# Autodesk Inventor assembly: BombaPerisImprimible
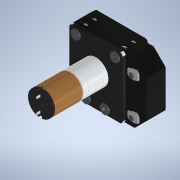
[picture p0: Inventor's stored thumbnail of the model, 180x180]
Saved by Autodesk Inventor 2020.2 (Build 242310000, 310)
## iProperties
Created: 2020-12-04
Part Number: BombaPerisImprimible
Document SubType Name: Assembly
Designer: JK
Sending System: Autodesk Inventor 2020
Preprocessor: ST-DEVELOPER v18
Title: D:\Desk\Drés\2020\Trabajo personal\jk\Podasana\bomba peristaltica\imp\BombaPerisImprimible.stp
Author: andre
## Documents named in this file (12)
- C:\Users\JK\Documents\Inventor\BioMixer\BombaPeristaltica\BombaPeristaltica.iam
- C:\Users\JK\Documents\Inventor\BioMixer\BombaPeristaltica\Impulsor.iam
- C:\Users\JK\Documents\Inventor\BioMixer\BombaPeristaltica\Caja.ipt
- C:\Users\JK\Documents\Inventor\BioMixer\BombaPeristaltica\TapaInferior.ipt
- C:\Users\JK\Documents\Inventor\BioMixer\BombaPeristaltica\TapaSuperior.ipt
- C:\Users\JK\Documents\Inventor\BioMixer\BombaPeristaltica\PernoM3x6Avellanado.ipt
- C:\Users\JK\Documents\Inventor\BioMixer\BombaPeristaltica\PernoM5x25Plano.ipt
- C:\Users\JK\Documents\Inventor\BioMixer\BombaPeristaltica\PernoM5x10Plano.ipt
- C:\Users\JK\Documents\Inventor\BioMixer\BombaPeristaltica\TuercaTM5Perfil2020.ipt
- C:\Users\JK\Documents\Inventor\BioMixer\BombaPeristaltica\MotorDC12V100RPM.ipt
- C:\Users\JK\Documents\Inventor\BioMixer\BombaPeristaltica\TuercaM5.ipt
- C:\Users\JK\Documents\Inventor\BioMixer\BombaPeristaltica\GolillaM5DIN125.ipt
## Components (28 placed, 11 different names)
1. MotorDC12V100RPM:1
2. Impulsor [sub-assembly] — Mate:67
3. Caja — Mate:3, Mate:4, Mate:16, Mate:19, Mate:24, Mate:25, Mate:26, Mate:27, Mate:35, Mate:48, Mate:49, Mate:50, Mate:51, Mate:52, Mate:53, Mate:54, Mate:55, Mate:56, Angle:1
4. TapaSuperior — Mate:3, Mate:4, Mate:38, Mate:39, Mate:40, Mate:41, Mate:42
5. PernoM5x10Plano:1 — Flush:13, Flush:14, Mate:40, Mate:58
6. PernoM5x10Plano:2 — Flush:13, Mate:41, Mate:42, Mate:60
7. PernoM5x10Plano:3 — Flush:15, Mate:38, Mate:56, Mate:63
8. PernoM5x10Plano:4 — Flush:14, Flush:15, Mate:39, Mate:62
9. PernoM5x10Plano:5 — Flush:17, Flush:18, Mate:43, Mate:44, Mate:59
10. PernoM5x10Plano:6 — Flush:17, Mate:45, Mate:57
11. PernoM5x10Plano:7 — Flush:16, Mate:47, Mate:64
12. PernoM5x10Plano:8 — Flush:16, Flush:18, Mate:46, Mate:61
13. PernoM3x6Avellanado:1 — Flush:10
14. TapaInferior:1 — Mate:16, Mate:19, Flush:12, Mate:43, Mate:44, Mate:45, Mate:46, Mate:47, Mate:66
15. PernoM5x25Plano:1 — Mate:25, Mate:26, Mate:29, Flush:9
16. PernoM5x25Plano:2 — Mate:24, Mate:27, Mate:28, Flush:9
17. TuercaTM5Perfil2020:1 — Mate:28, Flush:8, Flush:11
18. TuercaTM5Perfil2020:2 — Mate:29, Flush:8, Mate:35, Flush:11
19. PernoM3x6Avellanado:2 — Flush:10, Flush:12
20. TuercaM5:1 — Mate:48, Angle:7, Mate:63
21. TuercaM5:2 — Mate:49, Angle:5, Mate:62
22. TuercaM5:3 — Mate:50, Angle:5, Angle:6, Mate:61
23. TuercaM5:4 — Mate:51, Angle:6, Angle:7, Mate:64
24. TuercaM5:5 — Mate:52, Angle:4, Mate:60
25. TuercaM5:6 — Mate:55, Angle:2, Angle:3, Mate:58
26. TuercaM5:7 — Mate:54, Mate:57, Angle:1, Angle:2
27. TuercaM5:8 — Mate:53, Angle:3, Angle:4, Mate:59
28. GolillaM5DIN125:1 — Mate:66, Mate:67
## Relationships (65: Mate 47, Flush 11, Angle 7)
- Mate:3: Caja ↔ TapaSuperior
- Mate:4: Caja ↔ TapaSuperior
- Mate:16: Caja ↔ TapaInferior:1
- Mate:19: Caja ↔ TapaInferior:1
- Mate:24: Caja ↔ PernoM5x25Plano:2
- Mate:25: Caja ↔ PernoM5x25Plano:1
- Mate:26: Caja ↔ PernoM5x25Plano:1
- Mate:27: Caja ↔ PernoM5x25Plano:2
- Mate:28: PernoM5x25Plano:2 ↔ TuercaTM5Perfil2020:1
- Mate:29: PernoM5x25Plano:1 ↔ TuercaTM5Perfil2020:2
- Flush:8: TuercaTM5Perfil2020:1 ↔ TuercaTM5Perfil2020:2
- Flush:9: PernoM5x25Plano:1 ↔ PernoM5x25Plano:2
- [Mate]: MotorDC12V100RPM:1 ↔ TapaInferior:1
- [Mate]: MotorDC12V100RPM:1 ↔ TapaInferior:1
- [Mate]: MotorDC12V100RPM:1 ↔ PernoM3x6Avellanado:1
- [Mate]: MotorDC12V100RPM:1 ↔ PernoM3x6Avellanado:2
- Flush:10: PernoM3x6Avellanado:1 ↔ PernoM3x6Avellanado:2
- Mate:35 (1 mm): Caja ↔ TuercaTM5Perfil2020:2
- Flush:11: TuercaTM5Perfil2020:1 ↔ TuercaTM5Perfil2020:2
- Flush:12: TapaInferior:1 ↔ PernoM3x6Avellanado:2
- [Mate]: MotorDC12V100RPM:1 ↔ TapaInferior:1
- [Mate]: MotorDC12V100RPM:1 ↔ Impulsor
- Flush:13: PernoM5x10Plano:1 ↔ PernoM5x10Plano:2
- Flush:14: PernoM5x10Plano:1 ↔ PernoM5x10Plano:4
- Flush:15: PernoM5x10Plano:3 ↔ PernoM5x10Plano:4
- Mate:38: TapaSuperior ↔ PernoM5x10Plano:3
- Mate:39: TapaSuperior ↔ PernoM5x10Plano:4
- Mate:40: TapaSuperior ↔ PernoM5x10Plano:1
- Mate:41: TapaSuperior ↔ PernoM5x10Plano:2
- Mate:42: TapaSuperior ↔ PernoM5x10Plano:2
- Flush:16: PernoM5x10Plano:7 ↔ PernoM5x10Plano:8
- Flush:17: PernoM5x10Plano:5 ↔ PernoM5x10Plano:6
- Flush:18: PernoM5x10Plano:5 ↔ PernoM5x10Plano:8
- Mate:43: PernoM5x10Plano:5 ↔ TapaInferior:1
- Mate:44: PernoM5x10Plano:5 ↔ TapaInferior:1
- Mate:45: PernoM5x10Plano:6 ↔ TapaInferior:1
- Mate:46: PernoM5x10Plano:8 ↔ TapaInferior:1
- Mate:47: PernoM5x10Plano:7 ↔ TapaInferior:1
- Mate:48: Caja ↔ TuercaM5:1
- Mate:49: Caja ↔ TuercaM5:2
- Mate:50: Caja ↔ TuercaM5:3
- Mate:51: Caja ↔ TuercaM5:4
- Mate:52: Caja ↔ TuercaM5:5
- Mate:53: Caja ↔ TuercaM5:8
- Mate:54: Caja ↔ TuercaM5:7
- Mate:55: Caja ↔ TuercaM5:6
- Mate:56: Caja ↔ PernoM5x10Plano:3
- Mate:57: PernoM5x10Plano:6 ↔ TuercaM5:7
- Angle:1 (0 deg): Caja ↔ TuercaM5:7
- Angle:2 (0 deg): TuercaM5:6 ↔ TuercaM5:7
- Angle:3 (0 deg): TuercaM5:6 ↔ TuercaM5:8
- Angle:4 (0 deg): TuercaM5:5 ↔ TuercaM5:8
- Mate:58: PernoM5x10Plano:1 ↔ TuercaM5:6
- Mate:59: PernoM5x10Plano:5 ↔ TuercaM5:8
- Mate:60: PernoM5x10Plano:2 ↔ TuercaM5:5
- Angle:5 (0 deg): TuercaM5:2 ↔ TuercaM5:3
- Angle:6 (0 deg): TuercaM5:3 ↔ TuercaM5:4
- Angle:7 (0 deg): TuercaM5:1 ↔ TuercaM5:4
- Mate:61: PernoM5x10Plano:8 ↔ TuercaM5:3
- Mate:62: PernoM5x10Plano:4 ↔ TuercaM5:2
- Mate:63: PernoM5x10Plano:3 ↔ TuercaM5:1
- Mate:64: PernoM5x10Plano:7 ↔ TuercaM5:4
- [Mate]: MotorDC12V100RPM:1 ↔ GolillaM5DIN125:1
- Mate:66: TapaInferior:1 ↔ GolillaM5DIN125:1
- Mate:67: Impulsor ↔ GolillaM5DIN125:1
